# Autodesk Inventor assembly: Assembly2
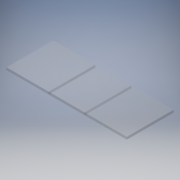
[picture p0: Inventor's stored thumbnail of the model, 180x180]
Saved by Autodesk Inventor 2017 (Build 210142000, 142)
## iProperties
Created: 2016-08-19
Part Number: Assembly2
Document SubType Name: Assembly
Designer: Alunos
Author: Alunos
## Documents named in this file (3)
- D:\ARQUIVOS\Arquivos\4º termo\TCC\TCC\Assembly2.iam
- D:\ARQUIVOS\Arquivos\4º termo\TCC\TCC\Frente-inferior-E-D.ipt
- D:\ARQUIVOS\Arquivos\4º termo\TCC\TCC\Frente inferior - porta1.ipt
## Components (3 placed, 2 different names)
1. Frente-inferior-E-D:1 — Rigid:1
2. Frente-inferior-E-D:2 — Rigid:2
3. Frente inferior - porta1:1 — Rigid:1, Rigid:2
## Relationships (2: WeldJoint 2)
- Rigid:1 [WeldJoint]: Frente-inferior-E-D:1 ↔ Frente inferior - porta1:1
- Rigid:2 [WeldJoint]: Frente-inferior-E-D:2 ↔ Frente inferior - porta1:1
